# Autodesk Inventor assembly: Chassis frame
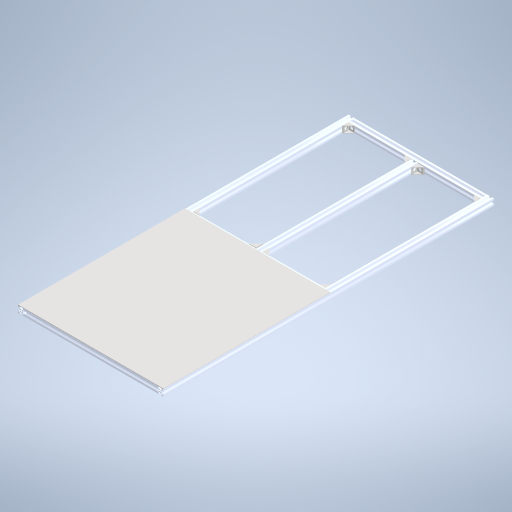
[picture p0: Inventor's stored thumbnail of the model, 512x512]
Saved by Autodesk Inventor 2023.1 (Build 271208000, 208)
## iProperties
Created: 2023-01-21
Part Number: Chassis frame
Document SubType Name: Assembly
Designer: eplym
Author: eplym
## Documents named in this file (7)
- C:\Users\eplym\Downloads\Chassis frame.iam
- C:\Users\eplym\Downloads\T-Slot 1m.ipt
- C:\Users\eplym\Downloads\T-Slot frame.ipt
- C:\Users\eplym\Downloads\T-Slot spine.ipt
- C:\Users\eplym\Downloads\T-Slot rib.ipt
- C:\Users\eplym\Downloads\sheet.ipt
- C:\Users\eplym\Downloads\corner bracket.ipt
## Components (24 placed, 6 different names)
1. T-Slot 1m:1 — Mate:1, Flush:3, Flush:4, Mate:19, Mate:20, Mate:33, Mate:35
2. T-Slot 1m:2 — Mate:2, Mate:3, Flush:1, Flush:2, Mate:7, Flush:6, Flush:9, Mate:12, Mate:27, Mate:29, Mate:43
3. T-Slot frame:1 — Mate:1, Mate:2, Flush:1, Flush:2, Flush:4, Mate:11, Flush:5, Flush:7, Flush:8, Flush:10, Mate:13, Mate:14, Mate:17, Mate:18
4. T-Slot frame:2 — Mate:3, Mate:4, Flush:3, Mate:9, Mate:10, Mate:34, Mate:36, Mate:41, Mate:42
5. T-Slot spine:1 — Mate:4, Mate:5, Mate:6, Mate:8, Mate:15, Mate:16, Mate:23, Mate:24, Mate:30, Mate:37, Mate:38, Mate:40
6. T-Slot rib:1 — Mate:5, Mate:7, Mate:8, Mate:9, Mate:25, Mate:26, Mate:28, Mate:31
7. T-Slot rib:2 — Mate:6, Mate:10, Mate:21, Mate:22, Mate:32, Mate:39
8. sheet:1 — Mate:11, Flush:5, Flush:6, Flush:7, Flush:8, Flush:9, Flush:10
9. corner bracket:1 — Mate:30, Mate:31
10. corner bracket:2 — Mate:32, Mate:33
11. corner bracket:3 — Mate:26, Mate:27
12. corner bracket:4 — Mate:24, Mate:25
13. corner bracket:5 — Mate:28, Mate:29
14. corner bracket:6 — Mate:34, Mate:35
15. corner bracket:7 — Mate:22, Mate:23
16. corner bracket:8 — Mate:20, Mate:21
17. corner bracket:9 — Mate:18, Mate:19
18. corner bracket:10 — Mate:14, Mate:15
19. corner bracket:11 — Mate:16, Mate:17
20. corner bracket:12 — Mate:12, Mate:13
21. corner bracket:13 — Mate:42, Mate:43
22. corner bracket:14 — Mate:38, Mate:39
23. corner bracket:15 — Mate:40, Mate:41
24. corner bracket:16 — Mate:36, Mate:37
## Relationships (53: Mate 43, Flush 10)
- Mate:1: T-Slot 1m:1 ↔ T-Slot frame:1
- Mate:2: T-Slot 1m:2 ↔ T-Slot frame:1
- Mate:3: T-Slot 1m:2 ↔ T-Slot frame:2
- Mate:4: T-Slot frame:2 ↔ T-Slot spine:1
- Flush:1: T-Slot 1m:2 ↔ T-Slot frame:1
- Flush:2: T-Slot 1m:2 ↔ T-Slot frame:1
- Flush:3: T-Slot 1m:1 ↔ T-Slot frame:2
- Flush:4: T-Slot 1m:1 ↔ T-Slot frame:1
- Mate:5: T-Slot spine:1 ↔ T-Slot rib:1
- Mate:6: T-Slot spine:1 ↔ T-Slot rib:2
- Mate:7: T-Slot 1m:2 ↔ T-Slot rib:1
- Mate:8: T-Slot spine:1 ↔ T-Slot rib:1
- Mate:9 (470 mm): T-Slot frame:2 ↔ T-Slot rib:1
- Mate:10 (470 mm): T-Slot frame:2 ↔ T-Slot rib:2
- Mate:11: T-Slot frame:1 ↔ sheet:1
- Flush:5: T-Slot frame:1 ↔ sheet:1
- Flush:6: T-Slot 1m:2 ↔ sheet:1
- Flush:7: T-Slot frame:1 ↔ sheet:1
- Flush:8: T-Slot frame:1 ↔ sheet:1
- Flush:9: T-Slot 1m:2 ↔ sheet:1
- Flush:10: T-Slot frame:1 ↔ sheet:1
- Mate:12: T-Slot 1m:2 ↔ corner bracket:12
- Mate:13: T-Slot frame:1 ↔ corner bracket:12
- Mate:14: T-Slot frame:1 ↔ corner bracket:10
- Mate:15: T-Slot spine:1 ↔ corner bracket:10
- Mate:16: T-Slot spine:1 ↔ corner bracket:11
- Mate:17: T-Slot frame:1 ↔ corner bracket:11
- Mate:18: T-Slot frame:1 ↔ corner bracket:9
- Mate:19: T-Slot 1m:1 ↔ corner bracket:9
- Mate:20: T-Slot 1m:1 ↔ corner bracket:8
- Mate:21: T-Slot rib:2 ↔ corner bracket:8
- Mate:22: T-Slot rib:2 ↔ corner bracket:7
- Mate:23: T-Slot spine:1 ↔ corner bracket:7
- Mate:24: T-Slot spine:1 ↔ corner bracket:4
- Mate:25: T-Slot rib:1 ↔ corner bracket:4
- Mate:26: T-Slot rib:1 ↔ corner bracket:3
- Mate:27: T-Slot 1m:2 ↔ corner bracket:3
- Mate:28: T-Slot rib:1 ↔ corner bracket:5
- Mate:29: T-Slot 1m:2 ↔ corner bracket:5
- Mate:30: T-Slot spine:1 ↔ corner bracket:1
- Mate:31: T-Slot rib:1 ↔ corner bracket:1
- Mate:32: T-Slot rib:2 ↔ corner bracket:2
- Mate:33: T-Slot 1m:1 ↔ corner bracket:2
- Mate:34: T-Slot frame:2 ↔ corner bracket:6
- Mate:35: T-Slot 1m:1 ↔ corner bracket:6
- Mate:36: T-Slot frame:2 ↔ corner bracket:16
- Mate:37: T-Slot spine:1 ↔ corner bracket:16
- Mate:38: T-Slot spine:1 ↔ corner bracket:14
- Mate:39: T-Slot rib:2 ↔ corner bracket:14
- Mate:40: T-Slot spine:1 ↔ corner bracket:15
- Mate:41: T-Slot frame:2 ↔ corner bracket:15
- Mate:42: T-Slot frame:2 ↔ corner bracket:13
- Mate:43: T-Slot 1m:2 ↔ corner bracket:13
